# Autodesk Inventor assembly: hodinky-assembly2
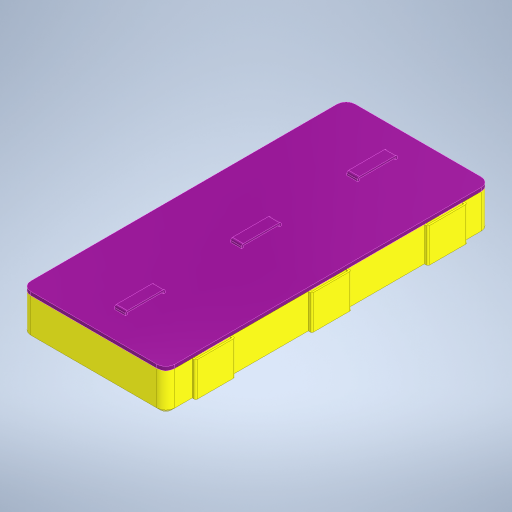
[picture p0: Inventor's stored thumbnail of the model, 512x512]
Saved by Autodesk Inventor 2023.2 (Build 272271000, 271)
## iProperties
Created: 2024-02-06
Part Number: hodinky-assembly2
Document SubType Name: Assembly
Designer: marek
Author: marek
## Documents named in this file (3)
- C:\Users\marek\Documents\Martin\hodinky-assembly2.iam
- C:\Users\marek\Documents\Martin\hodinky3-horní.ipt
- C:\Users\marek\Documents\Martin\hodinky4.ipt
## Components (2 placed, 2 different names)
1. hodinky3-horní:1 — Mate:1, Mate:2
2. hodinky4:1 — Mate:1, Mate:2, Mate:3, Mate:4, Flush:1
## Relationships (5: Mate 4, Flush 1)
- Mate:1: hodinky3-horní:1 ↔ hodinky4:1
- Mate:2: hodinky3-horní:1 ↔ hodinky4:1
- Mate:3: hodinky4:1
- Mate:4: hodinky4:1
- Flush:1: hodinky4:1
